# Autodesk Inventor assembly: clamp_L50
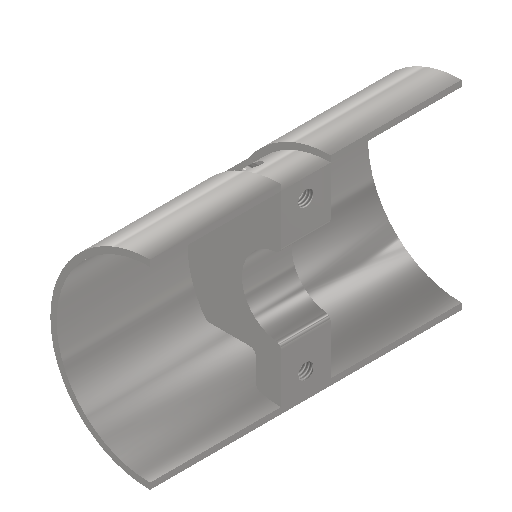
[picture p0: Inventor's stored thumbnail of the model, 512x512]
Saved by Autodesk Inventor 2026.2 (Build 302298000, 298)
## iProperties
Created: 2025-10-23
Part Number: clamp_L50
Document SubType Name: Assembly
Designer: jin20
Author: jin20
## Documents named in this file (3)
- D:\repos\PIHTI\SpectroscopySystem_Hayashi\Probe\clamp_L50.iam
- D:\repos\PIHTI\SpectroscopySystem_Hayashi\Probe\clamp-ring.ipt
- D:\repos\PIHTI\SpectroscopySystem_Hayashi\Probe\cover-pipe_L50.ipt
## Components (2 placed, 2 different names)
1. clamp-ring:1 — 挿入:1
2. cover-pipe_L50:1 — 挿入:1
## Relationships (1: Insert 1)
- 挿入:1 [Insert]: clamp-ring:1 ↔ cover-pipe_L50:1
